# Autodesk Inventor assembly: BaseMini
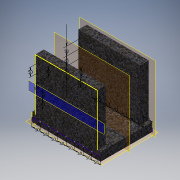
[picture p0: Inventor's stored thumbnail of the model, 180x180]
Saved by Autodesk Inventor 2016 (Build 200138000, 138)
## iProperties
Created: 2015-08-01
Part Number: BaseMini
Document SubType Name: Assembly
Designer: myhome
Author: myhome
## Documents named in this file (3)
- C:\Users\myhome\Documents\Inventor\Printer\EpoxyGraniteBase\BaseMini.iam
- C:\Users\myhome\Documents\Inventor\Printer\EpoxyGraniteBase\BaseMini.ipt
- C:\Users\myhome\Documents\Inventor\Content Center Files\R2016\en-US\U 2605\Unbrako - M4 x  40(5).ipt
## Components (27 placed, 2 different names)
1. BaseMini:1 — Flush:1, Flush:2, Flush:3, Rotational:1, Rotational:2, Rotational:3, Rotational:4, Rotational:5, Rotational:6, Rotational:7, Rotational:17, Rotational:18, Rotational:19, Rotational:8, Rotational:9, Rotational:10, Rotational:11, Rotational:20, Rotational:12, Rotational:13, Rotational:21, Rotational:22, Rigid:7, Rigid:8, Rigid:9, Rigid:10, Rigid:11, Rotational:15, Rotational:16
2. Unbrako Hex Socket Button Cap - Metric M4 x 40:1 — Rotational:1
3. Unbrako Hex Socket Button Cap - Metric M4 x 40:2 — Rotational:2
4. Unbrako Hex Socket Button Cap - Metric M4 x 40:3 — Rotational:3
5. Unbrako Hex Socket Button Cap - Metric M4 x 40:4 — Rotational:4
6. Unbrako Hex Socket Button Cap - Metric M4 x 40:6 — Rotational:5
7. Unbrako Hex Socket Button Cap - Metric M4 x 40:7 — Rotational:6
8. Unbrako Hex Socket Button Cap - Metric M4 x 40:8 — Rotational:7
9. Unbrako Hex Socket Button Cap - Metric M4 x 40:9 — Rotational:10
10. Unbrako Hex Socket Button Cap - Metric M4 x 40:10 — Rotational:8
11. Unbrako Hex Socket Button Cap - Metric M4 x 40:12 — Rotational:17
12. Unbrako Hex Socket Button Cap - Metric M4 x 40:14 — Rotational:19
13. Unbrako Hex Socket Button Cap - Metric M4 x 40:16 — Rotational:9
14. Unbrako Hex Socket Button Cap - Metric M4 x 40:17 — Rotational:11
15. Unbrako Hex Socket Button Cap - Metric M4 x 40:18 — Rotational:18
16. Unbrako Hex Socket Button Cap - Metric M4 x 40:19 — Rotational:12
17. Unbrako Hex Socket Button Cap - Metric M4 x 40:20 — Rigid:11
18. Unbrako Hex Socket Button Cap - Metric M4 x 40:21 — Rigid:10
19. Unbrako Hex Socket Button Cap - Metric M4 x 40:22 — Rigid:9
20. Unbrako Hex Socket Button Cap - Metric M4 x 40:23 — Rotational:20
21. Unbrako Hex Socket Button Cap - Metric M4 x 40:24 — Rotational:22
22. Unbrako Hex Socket Button Cap - Metric M4 x 40:25 — Rigid:8
23. Unbrako Hex Socket Button Cap - Metric M4 x 40:26 — Rigid:7
24. Unbrako Hex Socket Button Cap - Metric M4 x 40:27 — Rotational:21
25. Unbrako Hex Socket Button Cap - Metric M4 x 40:28 — Rotational:13
26. Unbrako Hex Socket Button Cap - Metric M4 x 40:29 — Rotational:15
27. Unbrako Hex Socket Button Cap - Metric M4 x 40:30 — Rotational:16
## Relationships (29: RevoluteJoint 21, WeldJoint 5, Flush 3)
- Flush:1: BaseMini:1
- Flush:2: BaseMini:1
- Flush:3: BaseMini:1
- Rotational:1 [RevoluteJoint]: BaseMini:1 ↔ Unbrako Hex Socket Button Cap - Metric M4 x 40:1
- Rotational:2 [RevoluteJoint]: BaseMini:1 ↔ Unbrako Hex Socket Button Cap - Metric M4 x 40:2
- Rotational:3 [RevoluteJoint]: BaseMini:1 ↔ Unbrako Hex Socket Button Cap - Metric M4 x 40:3
- Rotational:4 [RevoluteJoint]: BaseMini:1 ↔ Unbrako Hex Socket Button Cap - Metric M4 x 40:4
- Rotational:5 [RevoluteJoint]: BaseMini:1 ↔ Unbrako Hex Socket Button Cap - Metric M4 x 40:6
- Rotational:6 [RevoluteJoint]: BaseMini:1 ↔ Unbrako Hex Socket Button Cap - Metric M4 x 40:7
- Rotational:7 [RevoluteJoint]: BaseMini:1 ↔ Unbrako Hex Socket Button Cap - Metric M4 x 40:8
- Rotational:17 [RevoluteJoint]: BaseMini:1 ↔ Unbrako Hex Socket Button Cap - Metric M4 x 40:12
- Rotational:18 [RevoluteJoint]: BaseMini:1 ↔ Unbrako Hex Socket Button Cap - Metric M4 x 40:18
- Rotational:19 [RevoluteJoint]: BaseMini:1 ↔ Unbrako Hex Socket Button Cap - Metric M4 x 40:14
- Rotational:8 [RevoluteJoint]: BaseMini:1 ↔ Unbrako Hex Socket Button Cap - Metric M4 x 40:10
- Rotational:9 [RevoluteJoint]: BaseMini:1 ↔ Unbrako Hex Socket Button Cap - Metric M4 x 40:16
- Rotational:10 [RevoluteJoint]: BaseMini:1 ↔ Unbrako Hex Socket Button Cap - Metric M4 x 40:9
- Rotational:11 [RevoluteJoint]: BaseMini:1 ↔ Unbrako Hex Socket Button Cap - Metric M4 x 40:17
- Rotational:20 [RevoluteJoint]: BaseMini:1 ↔ Unbrako Hex Socket Button Cap - Metric M4 x 40:23
- Rotational:12 [RevoluteJoint]: BaseMini:1 ↔ Unbrako Hex Socket Button Cap - Metric M4 x 40:19
- Rotational:13 [RevoluteJoint]: BaseMini:1 ↔ Unbrako Hex Socket Button Cap - Metric M4 x 40:28
- Rotational:21 [RevoluteJoint]: BaseMini:1 ↔ Unbrako Hex Socket Button Cap - Metric M4 x 40:27
- Rotational:22 [RevoluteJoint]: BaseMini:1 ↔ Unbrako Hex Socket Button Cap - Metric M4 x 40:24
- Rigid:7 [WeldJoint]: BaseMini:1 ↔ Unbrako Hex Socket Button Cap - Metric M4 x 40:26
- Rigid:8 [WeldJoint]: BaseMini:1 ↔ Unbrako Hex Socket Button Cap - Metric M4 x 40:25
- Rigid:9 [WeldJoint]: BaseMini:1 ↔ Unbrako Hex Socket Button Cap - Metric M4 x 40:22
- Rigid:10 [WeldJoint]: BaseMini:1 ↔ Unbrako Hex Socket Button Cap - Metric M4 x 40:21
- Rigid:11 [WeldJoint]: BaseMini:1 ↔ Unbrako Hex Socket Button Cap - Metric M4 x 40:20
- Rotational:15 [RevoluteJoint]: BaseMini:1 ↔ Unbrako Hex Socket Button Cap - Metric M4 x 40:29
- Rotational:16 [RevoluteJoint]: BaseMini:1 ↔ Unbrako Hex Socket Button Cap - Metric M4 x 40:30
